# Autodesk Inventor assembly: Front A Battery Pack
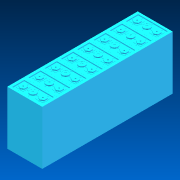
[picture p0: Inventor's stored thumbnail of the model, 180x180]
Saved by Autodesk Inventor 2012 (Build 160160000, 160)
## iProperties
Created: 2012-07-05
Part Number: Front A Battery Pack
Document SubType Name: Assembly
Designer: Hemant
Author: Hemant
## Documents named in this file (2)
- C:\Users\Hemant\Documents\Battery Boxes\Batteries\Front A Battery Pack.iam
- C:\Users\Hemant\Documents\Battery Boxes\Batteries\CALB100AH final.ipt
## Components (8 placed, 1 different names)
1. CALB100AH final:1
2. CALB100AH final:2
3. CALB100AH final:3
4. CALB100AH final:4
5. CALB100AH final:5
6. CALB100AH final:6
7. CALB100AH final:7
8. CALB100AH final:8
## Component patterns: (8 elements, first: CALB100AH final:1)
